# Autodesk Inventor assembly: assembly Medicijnenkluisje
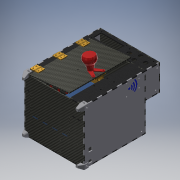
[picture p0: Inventor's stored thumbnail of the model, 180x180]
Saved by Autodesk Inventor 2019 (Build 230136000, 136)
## iProperties
Created: 2021-01-09
Part Number: assembly Medicijnenkluisje
Document SubType Name: Assembly
Designer: Stefan
Author: Stefan
## Documents named in this file (24)
- E:\project MS\1 github\assembly Medicijnenkluisje.iam
- E:\project MS\kast 3.1 achterplaat.ipt
- E:\project MS\kast 3.2 zij plaat.ipt
- E:\project MS\kast 3.3 boven onder plaat.ipt
- E:\project MS\bakjes legger.ipt
- E:\project MS\af\slot\pinhouder slot 2 d 4.ipt
- E:\project MS\plaatwerk\achterkant.ipt
- E:\project MS\plaatwerk\dunne cover plaat.ipt
- E:\project MS\plaatwerk 2\dikke cover plaat.ipt
- E:\project MS\plaatwerk\deur.ipt
- E:\project MS\scharnier 1.1 deel 2.ipt
- E:\project MS\scharnier 1.1 deel 1.ipt
- E:\project MS\af\slot\pinhouder slot d 2.ipt
- E:\project MS\af\slot\pinhouder slot d 1.ipt
- E:\project MS\plaatwerk 2\voorplaat.ipt
- E:\project MS\plaatwerk\zijplaat 3.ipt
- E:\project MS\plaatwerk\zijplaat RFID 2.ipt
- E:\project MS\plaatwerk\achterkant LCD.ipt
- E:\project MS\plaatwerk\LCD top.ipt
- E:\project MS\plaatwerk 2\kast onder plaat.ipt
- E:\project MS\afwerking\pootjes.ipt
- E:\project MS\einde ptroject\parts ipt\2 kanten verbinding voor.ipt
- E:\project MS\einde ptroject\parts ipt\3 kanten verbinding 1.ipt
- E:\project MS\einde ptroject\parts ipt\deurknop.ipt
## Components (48 placed, 23 different names)
1. kast 3.1 achterplaat:1 — Mate:1, Mate:2, Mate:3, Mate:4, Mate:5, Mate:6
2. kast 3.2 zij plaat:1 — Mate:1, Mate:3, Mate:5, Mate:7, Mate:8, Mate:9, Cylindrical:15, Cylindrical:16, Cylindrical:17, Cylindrical:18, Cylindrical:19, Cylindrical:20, Cylindrical:21, Cylindrical:22, Cylindrical:23, Cylindrical:24, Cylindrical:25, Cylindrical:26, Cylindrical:27, Cylindrical:28, Mate:33, Mate:34, Mate:35, Mate:36, Mate:37, Mate:38, Mate:39
3. kast 3.2 zij plaat:2 — Mate:2, Mate:4, Mate:6, Cylindrical:1, Cylindrical:2, Cylindrical:3, Cylindrical:4, Cylindrical:5, Cylindrical:6, Cylindrical:7, Cylindrical:8, Cylindrical:9, Cylindrical:10, Cylindrical:11, Cylindrical:12, Cylindrical:13, Cylindrical:14, Mate:26, Mate:27, Mate:28, Mate:29, Mate:30, Mate:31, Mate:32
4. bakjes legger:1 — Cylindrical:15, Cylindrical:22, Mate:39
5. bakjes legger:2 — Cylindrical:16, Cylindrical:23, Mate:38
6. bakjes legger:3 — Cylindrical:17, Cylindrical:24, Mate:37
7. bakjes legger:4 — Cylindrical:18, Cylindrical:25, Mate:36
8. bakjes legger:5 — Cylindrical:19, Cylindrical:26, Mate:35
9. bakjes legger:6 — Cylindrical:20, Cylindrical:27, Mate:34
10. bakjes legger:7 — Cylindrical:21, Cylindrical:28, Mate:33
11. bakjes legger:8 — Cylindrical:1, Cylindrical:2, Mate:26
12. bakjes legger:9 — Cylindrical:3, Cylindrical:4, Mate:27
13. bakjes legger:10 — Cylindrical:5, Cylindrical:6, Mate:28
14. bakjes legger:11 — Cylindrical:7, Cylindrical:8, Mate:29
15. bakjes legger:12 — Cylindrical:9, Cylindrical:10, Mate:30
16. bakjes legger:13 — Cylindrical:11, Cylindrical:12, Mate:31
17. bakjes legger:14 — Cylindrical:13, Cylindrical:14, Mate:32
18. pinhouder slot 2 d 4:1 — Mate:95, Mate:96, Mate:97
19. achterkant:1 — Mate:117, Mate:118, Mate:119, Mate:123, Mate:132, Mate:135, Mate:136, Mate:163, Mate:165
20. kast 3.3 boven onder plaat:1 — Mate:7, Mate:8, Mate:9, Mate:23, Mate:24, Mate:25, Mate:40, Mate:41, Mate:42, Mate:101, Mate:102, Mate:103, Mate:109, Mate:117, Mate:118, Mate:169, Mate:171
21. dunne cover plaat:1 — Mate:23, Mate:24, Mate:25
22. dikke cover plaat:1 — Mate:40, Mate:41, Mate:42
23. deur:1 — Mate:67, Mate:68, Mate:69, Mate:70, Mate:71, Mate:76, Mate:77, Mate:78, Mate:82, Mate:83, Mate:84, Mate:85, Mate:151, Mate:152, Mate:153
24. scharnier 1.1 deel 2:1 — Mate:55, Flush:1, Mate:70, Mate:82, Mate:84
25. scharnier 1.1 deel 2:2 — Mate:56, Flush:3, Mate:67, Mate:68, Mate:69
26. scharnier 1.1 deel 2:3 — Mate:57, Flush:2, Mate:71, Mate:83, Mate:85
27. scharnier 1.1 deel 1:1 — Mate:55, Flush:1, Mate:87, Mate:91, Mate:92
28. scharnier 1.1 deel 1:2 — Mate:56, Flush:3, Mate:86, Mate:89, Mate:90
29. scharnier 1.1 deel 1:3 — Mate:57, Flush:2, Mate:88, Mate:93, Mate:94
30. pinhouder slot d 2:1 — Mate:75, Flush:4, Flush:5, Mate:76
31. pinhouder slot d 1:1 — Mate:75, Flush:4, Flush:5, Mate:77, Mate:78
32. voorplaat:1 — Mate:86, Mate:87, Mate:88, Mate:89, Mate:90, Mate:91, Mate:92, Mate:93, Mate:94, Mate:95, Mate:96, Mate:97, Mate:104, Mate:105, Mate:106, Mate:107, Mate:108, Mate:125, Mate:127, Mate:128, Mate:129, Mate:145, Mate:149
33. deurknop:1 — Mate:151, Mate:152, Mate:153
34. zijplaat 3:1 — Mate:101, Mate:102, Mate:103, Mate:104, Mate:105, Mate:106, Mate:110, Mate:111, Mate:112, Mate:113, Mate:114, Mate:115, Mate:116, Mate:134, Mate:162, Mate:166
35. zijplaat RFID 2:1 — Mate:107, Mate:108, Mate:109, Mate:120, Mate:121, Mate:122, Mate:126, Mate:131, Mate:141, Mate:148, Mate:150, Mate:164
36. achterkant LCD:1 — Mate:110, Mate:111, Mate:112, Mate:140, Mate:167
37. LCD top:1 — Mate:114, Mate:115, Mate:116, Mate:139, Mate:146, Mate:147, Mate:168, Mate:170
38. kast onder plaat:1 — Mate:120, Mate:121, Mate:122, Mate:123, Mate:124, Mate:130, Mate:133
39. pootjes:1 — Mate:125, Mate:126, Mate:127
40. pootjes:2 — Mate:128, Mate:129, Mate:130
41. pootjes:3 — Mate:131, Mate:132, Mate:133
42. pootjes:4 — Mate:134, Mate:135, Mate:136
43. 2 kanten verbinding voor:1 — Mate:145, Mate:146, Mate:147
44. 3 kanten verbinding 1:1 — Mate:139, Mate:140, Mate:141, Mate:170
45. 2 kanten verbinding voor:2 — Mate:148, Mate:149, Mate:150
46. 3 kanten verbinding 1:2 — Mate:164, Mate:165, Mate:171
47. 3 kanten verbinding 1:3 — Mate:166, Mate:167, Mate:168
48. 3 kanten verbinding 1:4 — Mate:162, Mate:163, Mate:169
## Relationships (148: Mate 115, CylindricalJoint 28, Flush 5)
- Mate:1: kast 3.1 achterplaat:1 ↔ kast 3.2 zij plaat:1
- Mate:2: kast 3.1 achterplaat:1 ↔ kast 3.2 zij plaat:2
- Mate:3: kast 3.1 achterplaat:1 ↔ kast 3.2 zij plaat:1
- Mate:4: kast 3.1 achterplaat:1 ↔ kast 3.2 zij plaat:2
- Mate:5: kast 3.1 achterplaat:1 ↔ kast 3.2 zij plaat:1
- Mate:6: kast 3.1 achterplaat:1 ↔ kast 3.2 zij plaat:2
- Mate:7: kast 3.2 zij plaat:1 ↔ kast 3.3 boven onder plaat:1
- Mate:8: kast 3.2 zij plaat:1 ↔ kast 3.3 boven onder plaat:1
- Mate:9: kast 3.2 zij plaat:1 ↔ kast 3.3 boven onder plaat:1
- Cylindrical:1: kast 3.2 zij plaat:2 ↔ bakjes legger:8
- Cylindrical:2: kast 3.2 zij plaat:2 ↔ bakjes legger:8
- Cylindrical:3: kast 3.2 zij plaat:2 ↔ bakjes legger:9
- Cylindrical:4: kast 3.2 zij plaat:2 ↔ bakjes legger:9
- Cylindrical:5: kast 3.2 zij plaat:2 ↔ bakjes legger:10
- Cylindrical:6: kast 3.2 zij plaat:2 ↔ bakjes legger:10
- Cylindrical:7: kast 3.2 zij plaat:2 ↔ bakjes legger:11
- Cylindrical:8: kast 3.2 zij plaat:2 ↔ bakjes legger:11
- Cylindrical:9: kast 3.2 zij plaat:2 ↔ bakjes legger:12
- Cylindrical:10: kast 3.2 zij plaat:2 ↔ bakjes legger:12
- Cylindrical:11: kast 3.2 zij plaat:2 ↔ bakjes legger:13
- Cylindrical:12: kast 3.2 zij plaat:2 ↔ bakjes legger:13
- Cylindrical:13: kast 3.2 zij plaat:2 ↔ bakjes legger:14
- Cylindrical:14: kast 3.2 zij plaat:2 ↔ bakjes legger:14
- Cylindrical:15: kast 3.2 zij plaat:1 ↔ bakjes legger:1
- Cylindrical:16: kast 3.2 zij plaat:1 ↔ bakjes legger:2
- Cylindrical:17: kast 3.2 zij plaat:1 ↔ bakjes legger:3
- Cylindrical:18: kast 3.2 zij plaat:1 ↔ bakjes legger:4
- Cylindrical:19: kast 3.2 zij plaat:1 ↔ bakjes legger:5
- Cylindrical:20: kast 3.2 zij plaat:1 ↔ bakjes legger:6
- Cylindrical:21: kast 3.2 zij plaat:1 ↔ bakjes legger:7
- Cylindrical:22: kast 3.2 zij plaat:1 ↔ bakjes legger:1
- Cylindrical:23: kast 3.2 zij plaat:1 ↔ bakjes legger:2
- Cylindrical:24: kast 3.2 zij plaat:1 ↔ bakjes legger:3
- Cylindrical:25: kast 3.2 zij plaat:1 ↔ bakjes legger:4
- Cylindrical:26: kast 3.2 zij plaat:1 ↔ bakjes legger:5
- Cylindrical:27: kast 3.2 zij plaat:1 ↔ bakjes legger:6
- Cylindrical:28: kast 3.2 zij plaat:1 ↔ bakjes legger:7
- Mate:23: kast 3.3 boven onder plaat:1 ↔ dunne cover plaat:1
- Mate:24: kast 3.3 boven onder plaat:1 ↔ dunne cover plaat:1
- Mate:25: kast 3.3 boven onder plaat:1 ↔ dunne cover plaat:1
- Mate:26: kast 3.2 zij plaat:2 ↔ bakjes legger:8
- Mate:27: kast 3.2 zij plaat:2 ↔ bakjes legger:9
- Mate:28: kast 3.2 zij plaat:2 ↔ bakjes legger:10
- Mate:29: kast 3.2 zij plaat:2 ↔ bakjes legger:11
- Mate:30: kast 3.2 zij plaat:2 ↔ bakjes legger:12
- Mate:31: kast 3.2 zij plaat:2 ↔ bakjes legger:13
- Mate:32: kast 3.2 zij plaat:2 ↔ bakjes legger:14
- Mate:33: kast 3.2 zij plaat:1 ↔ bakjes legger:7
- Mate:34: kast 3.2 zij plaat:1 ↔ bakjes legger:6
- Mate:35: kast 3.2 zij plaat:1 ↔ bakjes legger:5
- Mate:36: kast 3.2 zij plaat:1 ↔ bakjes legger:4
- Mate:37: kast 3.2 zij plaat:1 ↔ bakjes legger:3
- Mate:38: kast 3.2 zij plaat:1 ↔ bakjes legger:2
- Mate:39: kast 3.2 zij plaat:1 ↔ bakjes legger:1
- Mate:40: kast 3.3 boven onder plaat:1 ↔ dikke cover plaat:1
- Mate:41: kast 3.3 boven onder plaat:1 ↔ dikke cover plaat:1
- Mate:42: kast 3.3 boven onder plaat:1 ↔ dikke cover plaat:1
- Mate:55: scharnier 1.1 deel 2:1 ↔ scharnier 1.1 deel 1:1
- Flush:1: scharnier 1.1 deel 2:1 ↔ scharnier 1.1 deel 1:1
- Mate:56: scharnier 1.1 deel 2:2 ↔ scharnier 1.1 deel 1:2
- Mate:57: scharnier 1.1 deel 2:3 ↔ scharnier 1.1 deel 1:3
- Flush:2: scharnier 1.1 deel 2:3 ↔ scharnier 1.1 deel 1:3
- Flush:3: scharnier 1.1 deel 2:2 ↔ scharnier 1.1 deel 1:2
- Mate:67: deur:1 ↔ scharnier 1.1 deel 2:2
- Mate:68: deur:1 ↔ scharnier 1.1 deel 2:2
- Mate:69: deur:1 ↔ scharnier 1.1 deel 2:2
- Mate:70: deur:1 ↔ scharnier 1.1 deel 2:1
- Mate:71: deur:1 ↔ scharnier 1.1 deel 2:3
- Mate:75: pinhouder slot d 2:1 ↔ pinhouder slot d 1:1
- Flush:4: pinhouder slot d 2:1 ↔ pinhouder slot d 1:1
- Flush:5: pinhouder slot d 2:1 ↔ pinhouder slot d 1:1
- Mate:76: deur:1 ↔ pinhouder slot d 2:1
- Mate:77: deur:1 ↔ pinhouder slot d 1:1
- Mate:78: deur:1 ↔ pinhouder slot d 1:1
- Mate:82: deur:1 ↔ scharnier 1.1 deel 2:1
- Mate:83: deur:1 ↔ scharnier 1.1 deel 2:3
- Mate:84: deur:1 ↔ scharnier 1.1 deel 2:1
- Mate:85: deur:1 ↔ scharnier 1.1 deel 2:3
- Mate:86: scharnier 1.1 deel 1:2 ↔ voorplaat:1
- Mate:87: scharnier 1.1 deel 1:1 ↔ voorplaat:1
- Mate:88: scharnier 1.1 deel 1:3 ↔ voorplaat:1
- Mate:89: scharnier 1.1 deel 1:2 ↔ voorplaat:1
- Mate:90: scharnier 1.1 deel 1:2 ↔ voorplaat:1
- Mate:91: scharnier 1.1 deel 1:1 ↔ voorplaat:1
- Mate:92: scharnier 1.1 deel 1:1 ↔ voorplaat:1
- Mate:93: scharnier 1.1 deel 1:3 ↔ voorplaat:1
- Mate:94: scharnier 1.1 deel 1:3 ↔ voorplaat:1
- Mate:95: pinhouder slot 2 d 4:1 ↔ voorplaat:1
- Mate:96: pinhouder slot 2 d 4:1 ↔ voorplaat:1
- Mate:97: pinhouder slot 2 d 4:1 ↔ voorplaat:1
- Mate:101: kast 3.3 boven onder plaat:1 ↔ zijplaat 3:1
- Mate:102: kast 3.3 boven onder plaat:1 ↔ zijplaat 3:1
- Mate:103: kast 3.3 boven onder plaat:1 ↔ zijplaat 3:1
- Mate:104: voorplaat:1 ↔ zijplaat 3:1
- Mate:105: voorplaat:1 ↔ zijplaat 3:1
- Mate:106: voorplaat:1 ↔ zijplaat 3:1
- Mate:107: voorplaat:1 ↔ zijplaat RFID 2:1
- Mate:108: voorplaat:1 ↔ zijplaat RFID 2:1
- Mate:109: kast 3.3 boven onder plaat:1 ↔ zijplaat RFID 2:1
- Mate:110: zijplaat 3:1 ↔ achterkant LCD:1
- Mate:111: zijplaat 3:1 ↔ achterkant LCD:1
- Mate:112: zijplaat 3:1 ↔ achterkant LCD:1
- Mate:113: zijplaat 3:1
- Mate:114: zijplaat 3:1 ↔ LCD top:1
- Mate:115: zijplaat 3:1 ↔ LCD top:1
- Mate:116: zijplaat 3:1 ↔ LCD top:1
- Mate:117: achterkant:1 ↔ kast 3.3 boven onder plaat:1
- Mate:118: achterkant:1 ↔ kast 3.3 boven onder plaat:1
- Mate:119: achterkant:1
- Mate:120: zijplaat RFID 2:1 ↔ kast onder plaat:1
- Mate:121: zijplaat RFID 2:1 ↔ kast onder plaat:1
- Mate:122: zijplaat RFID 2:1 ↔ kast onder plaat:1
- Mate:123: achterkant:1 ↔ kast onder plaat:1
- Mate:124: kast onder plaat:1
- Mate:125: voorplaat:1 ↔ pootjes:1
- Mate:126: zijplaat RFID 2:1 ↔ pootjes:1
- Mate:127: voorplaat:1 ↔ pootjes:1
- Mate:128: voorplaat:1 ↔ pootjes:2
- Mate:129: voorplaat:1 ↔ pootjes:2
- Mate:130: kast onder plaat:1 ↔ pootjes:2
- Mate:131: zijplaat RFID 2:1 ↔ pootjes:3
- Mate:132: achterkant:1 ↔ pootjes:3
- Mate:133: kast onder plaat:1 ↔ pootjes:3
- Mate:134: zijplaat 3:1 ↔ pootjes:4
- Mate:135: achterkant:1 ↔ pootjes:4
- Mate:136: achterkant:1 ↔ pootjes:4
- Mate:139: LCD top:1 ↔ 3 kanten verbinding 1:1
- Mate:140: achterkant LCD:1 ↔ 3 kanten verbinding 1:1
- Mate:141: zijplaat RFID 2:1 ↔ 3 kanten verbinding 1:1
- Mate:145: voorplaat:1 ↔ 2 kanten verbinding voor:1
- Mate:146: LCD top:1 ↔ 2 kanten verbinding voor:1
- Mate:147: LCD top:1 ↔ 2 kanten verbinding voor:1
- Mate:148: zijplaat RFID 2:1 ↔ 2 kanten verbinding voor:2
- Mate:149: voorplaat:1 ↔ 2 kanten verbinding voor:2
- Mate:150: zijplaat RFID 2:1 ↔ 2 kanten verbinding voor:2
- Mate:151: deur:1 ↔ deurknop:1
- Mate:152: deur:1 ↔ deurknop:1
- Mate:153: deur:1 ↔ deurknop:1
- Mate:162: zijplaat 3:1 ↔ 3 kanten verbinding 1:4
- Mate:163: achterkant:1 ↔ 3 kanten verbinding 1:4
- Mate:164: zijplaat RFID 2:1 ↔ 3 kanten verbinding 1:2
- Mate:165: achterkant:1 ↔ 3 kanten verbinding 1:2
- Mate:166: zijplaat 3:1 ↔ 3 kanten verbinding 1:3
- Mate:167: achterkant LCD:1 ↔ 3 kanten verbinding 1:3
- Mate:168: LCD top:1 ↔ 3 kanten verbinding 1:3
- Mate:169: kast 3.3 boven onder plaat:1 ↔ 3 kanten verbinding 1:4
- Mate:170: LCD top:1 ↔ 3 kanten verbinding 1:1
- Mate:171: kast 3.3 boven onder plaat:1 ↔ 3 kanten verbinding 1:2
